# Autodesk Inventor assembly: full_assembly
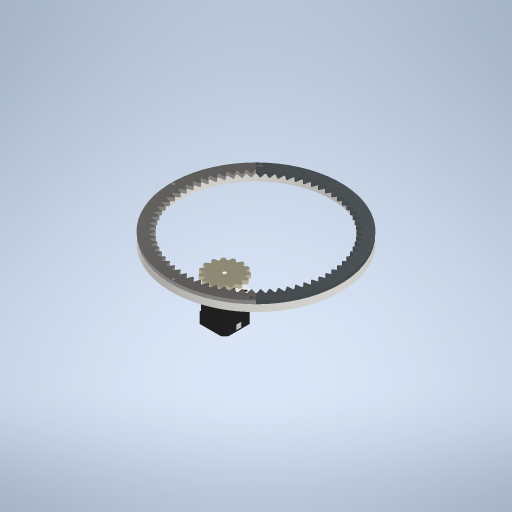
[picture p0: Inventor's stored thumbnail of the model, 512x512]
Saved by Autodesk Inventor 2023 (Build 270158000, 158)
## iProperties
Created: 2023-03-07
Part Number: full_assembly
Document SubType Name: Assembly
Designer: caleb
Author: caleb
## Documents named in this file (5)
- C:\Users\caleb\Documents\Inventor\SPICE\full_assembly.iam
- C:\Users\caleb\Documents\Inventor\SPICE\bearing_table.ipt
- C:\Users\caleb\Documents\Inventor\SPICE\bearing_gear.ipt
- C:\Users\caleb\Documents\Inventor\SPICE\motor.ipt
- C:\Users\caleb\Documents\Inventor\SPICE\motor_gear.ipt
## Components (5 placed, 4 different names)
1. bearing_table:1 — Mate:1, Mate:2, Mate:5, Mate:6
2. bearing_gear:1 — Mate:2, Mate:3, Mate:4, Mate:6
3. bearing_gear:2 — Mate:1, Mate:3, Mate:4, Mate:5, Flush:2
4. motor:1 — Mate:7, Flush:1, Mate:8
5. motor_gear:1 — Mate:7, Flush:1, Mate:8, Flush:2
## Relationships (10: Mate 8, Flush 2)
- Mate:1: bearing_table:1 ↔ bearing_gear:2
- Mate:2: bearing_table:1 ↔ bearing_gear:1
- Mate:3: bearing_gear:1 ↔ bearing_gear:2
- Mate:4: bearing_gear:1 ↔ bearing_gear:2
- Mate:5: bearing_table:1 ↔ bearing_gear:2
- Mate:6: bearing_table:1 ↔ bearing_gear:1
- Mate:7: motor:1 ↔ motor_gear:1
- Flush:1: motor:1 ↔ motor_gear:1
- Mate:8: motor:1 ↔ motor_gear:1
- Flush:2: bearing_gear:2 ↔ motor_gear:1
